# Autodesk Inventor assembly: Bottom Crossbrace
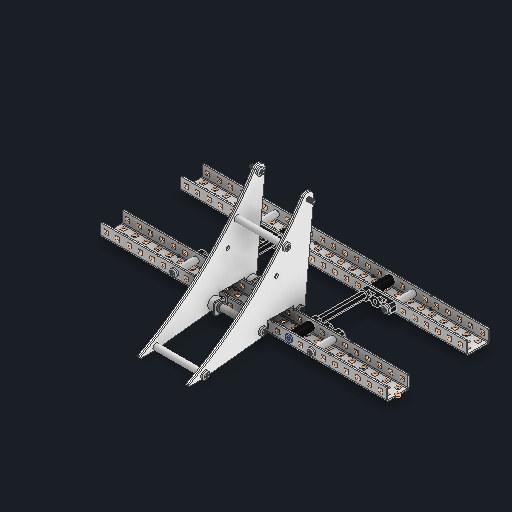
[picture p0: Inventor's stored thumbnail of the model, 512x512]
Saved by Autodesk Inventor 2025.1 (Build 291241000, 241)
## iProperties
Created: 2024-11-13
Part Number: Bottom Crossbrace
Document SubType Name: Assembly
Designer: avere
Author: avere
## Documents named in this file (5)
- C:\Users\avere\VEX\High Stakes\CAD\V3\Chassis\Structure\Bottom Crossbrace.iam
- C:\Users\avere\VEX\High Stakes\CAD\V3\Chassis\Structure\Front Crossbrace.iam
- C:\Users\avere\VEX\High Stakes\CAD\V3\Chassis\Structure\Mid Crossbrace.iam
- C:\Users\avere\VEX\High Stakes\CAD\ROBOPROS-CAD-Inventor\Structure\Standoff\Standoff 2.00.ipt
- C:\Users\avere\VEX\High Stakes\CAD\ROBOPROS-CAD-Inventor\Structure\Standoff.ipt
## Components (4 placed, 3 different names)
1. Front Crossbrace:1 [sub-assembly] — Insert:1, Mate:1
2. Mid Crossbrace:1 [sub-assembly] — Insert:2, Insert:3
3. Standoff 2.00:1 — Insert:3, Mate:1
4. Standoff 2.00:2 — Insert:1, Insert:2
## Relationships (4: Insert 3, Mate 1)
- Insert:1: Front Crossbrace:1 ↔ Standoff 2.00:2
- Insert:2: Mid Crossbrace:1 ↔ Standoff 2.00:2
- Insert:3: Mid Crossbrace:1 ↔ Standoff 2.00:1
- Mate:1: Front Crossbrace:1 ↔ Standoff 2.00:1
